# Autodesk Inventor assembly: sail(Midterm)
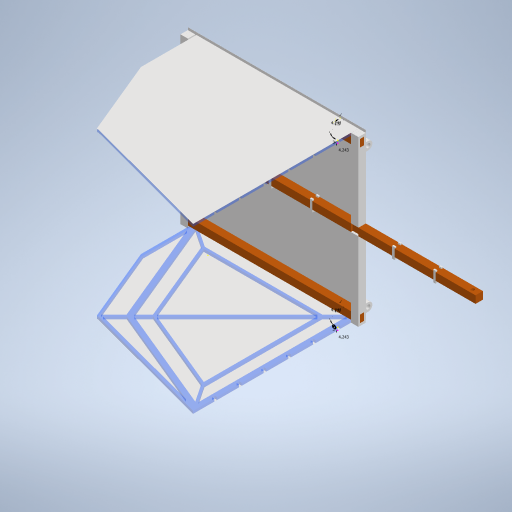
[picture p0: Inventor's stored thumbnail of the model, 512x512]
Saved by Autodesk Inventor 2024 (Build 280153000, 153)
## iProperties
Created: 2024-04-09
Part Number: sail(Midterm)
Document SubType Name: Assembly
Designer: USER
Author: USER
## Documents named in this file (11)
- E:\university\大三\大三下\機工實務\圖檔\DesignVer2\sail(Midterm).iam
- E:\university\大三\大三下\機工實務\圖檔\DesignVer2\main_Bar.ipt
- E:\university\大三\大三下\機工實務\圖檔\DesignVer2\main_Bar_3.ipt
- E:\university\大三\大三下\機工實務\圖檔\DesignVer2\Lower_Bar.ipt
- E:\university\大三\大三下\機工實務\圖檔\DesignVer2\upper_Bar.ipt
- E:\university\大三\大三下\機工實務\圖檔\DesignVer2\upper_Bar_3.ipt
- E:\university\大三\大三下\機工實務\圖檔\DesignVer2\side_Bar.ipt
- E:\university\大三\大三下\機工實務\圖檔\DesignVer2\side_sail.ipt
- E:\university\大三\大三下\機工實務\圖檔\DesignVer2\夾持器.ipt
- E:\university\大三\大三下\機工實務\圖檔\DesignVer2\帆布.ipt
- E:\university\大三\大三下\機工實務\圖檔\DesignVer2\帆布_中間.ipt
## Components (25 placed, 10 different names)
1. main_Bar:1 — 齊平:1, 齊平:2, 貼合:2, 貼合:7, 貼合:11, 貼合:26, 貼合:27, 貼合:28, 貼合:29, 貼合:33
2. main_Bar:2 — 齊平:1, 齊平:2, 齊平:3, 齊平:4, 貼合:1, 貼合:2, 貼合:5, 貼合:6, 貼合:30, 貼合:31, 貼合:32
3. main_Bar_3:1 — 齊平:3, 齊平:4, 貼合:1, 貼合:10, 齊平:13
4. Lower_Bar:1 — 齊平:5, 貼合:4, 齊平:8
5. Lower_Bar:2 — 齊平:5, 齊平:6, 貼合:3, 貼合:4, 齊平:7, 齊平:8
6. upper_Bar:1 — 貼合:9, 齊平:10, 齊平:11, 貼合:10
7. upper_Bar:2 — 貼合:8, 貼合:9, 齊平:9, 齊平:10, 齊平:11, 齊平:12, 齊平:13
8. upper_Bar_3:1 — 貼合:8, 齊平:9, 齊平:12, 貼合:11, 齊平:33
9. Lower_Bar:3 — 齊平:6, 貼合:3, 齊平:7, 貼合:5, 貼合:6, 貼合:7, 貼合:16, 貼合:17, 貼合:18, 貼合:19, 貼合:20, 貼合:21, 貼合:22, 貼合:24
10. side_Bar:1 — 貼合:12, 齊平:14, 齊平:17, 貼合:21, 齊平:22, 貼合:23, 齊平:32
11. side_Bar:2 — 貼合:12, 貼合:13, 齊平:14, 齊平:15, 齊平:16, 齊平:17, 貼合:20
12. side_Bar:3 — 貼合:13, 齊平:15, 齊平:16, 貼合:19
13. side_Bar:4 — 齊平:18, 齊平:20, 貼合:14
14. side_Bar:5 — 齊平:18, 齊平:19, 齊平:20, 齊平:21, 貼合:14, 貼合:15, 貼合:16, 貼合:18, 齊平:23
15. side_Bar:6 — 齊平:19, 齊平:21, 貼合:15, 貼合:17, 貼合:25
16. side_sail:1 — 齊平:22, 貼合:22, 貼合:23, 齊平:34, 齊平:36, 貼合:34
17. side_sail:2 — 齊平:23, 貼合:24, 貼合:25, 貼合:35, 齊平:37
18. 夾持器:1 — 齊平:24, 齊平:28, 齊平:29, 貼合:32
19. 夾持器:2 — 齊平:24, 齊平:25, 齊平:30, 貼合:31
20. 夾持器:3 — 齊平:25, 齊平:26, 齊平:31, 貼合:27, 貼合:28
21. 夾持器:4 — 齊平:26, 齊平:27, 齊平:29, 齊平:30, 齊平:31, 貼合:30
22. 夾持器:5 — 齊平:27, 貼合:26, 齊平:28, 貼合:29
23. 帆布:1 — 角度:1, 齊平:34, 齊平:35, 齊平:36, 貼合:34
24. 帆布_中間:1 — 貼合:33, 齊平:32, 齊平:33
25. 帆布:2 — 角度:1, 齊平:35, 貼合:35, 齊平:37
## Relationships (73: Flush 37, Mate 35, Angle 1)
- 齊平:1 [Flush]: main_Bar:1 ↔ main_Bar:2
- 齊平:2 [Flush]: main_Bar:1 ↔ main_Bar:2
- 齊平:3 [Flush]: main_Bar:2 ↔ main_Bar_3:1
- 齊平:4 [Flush]: main_Bar:2 ↔ main_Bar_3:1
- 貼合:1 [Mate]: main_Bar:2 ↔ main_Bar_3:1
- 貼合:2 [Mate]: main_Bar:1 ↔ main_Bar:2
- 齊平:5 [Flush]: Lower_Bar:1 ↔ Lower_Bar:2
- 齊平:6 [Flush]: Lower_Bar:2 ↔ Lower_Bar:3
- 貼合:3 [Mate]: Lower_Bar:2 ↔ Lower_Bar:3
- 貼合:4 [Mate]: Lower_Bar:1 ↔ Lower_Bar:2
- 齊平:7 [Flush]: Lower_Bar:2 ↔ Lower_Bar:3
- 齊平:8 [Flush]: Lower_Bar:1 ↔ Lower_Bar:2
- 貼合:5 [Mate]: main_Bar:2 ↔ Lower_Bar:3
- 貼合:6 [Mate]: main_Bar:2 ↔ Lower_Bar:3
- 貼合:7 [Mate]: main_Bar:1 ↔ Lower_Bar:3
- 貼合:8 [Mate]: upper_Bar:2 ↔ upper_Bar_3:1
- 貼合:9 [Mate]: upper_Bar:1 ↔ upper_Bar:2
- 齊平:9 [Flush]: upper_Bar:2 ↔ upper_Bar_3:1
- 齊平:10 [Flush]: upper_Bar:1 ↔ upper_Bar:2
- 齊平:11 [Flush]: upper_Bar:1 ↔ upper_Bar:2
- 齊平:12 [Flush]: upper_Bar:2 ↔ upper_Bar_3:1
- 貼合:10 [Mate]: main_Bar_3:1 ↔ upper_Bar:1
- 齊平:13 [Flush]: main_Bar_3:1 ↔ upper_Bar:2
- 貼合:11 [Mate]: main_Bar:1 ↔ upper_Bar_3:1
- 貼合:12 [Mate]: side_Bar:1 ↔ side_Bar:2
- 貼合:13 [Mate]: side_Bar:2 ↔ side_Bar:3
- 齊平:14 [Flush]: side_Bar:1 ↔ side_Bar:2
- 齊平:15 [Flush]: side_Bar:2 ↔ side_Bar:3
- 齊平:16 [Flush]: side_Bar:2 ↔ side_Bar:3
- 齊平:17 [Flush]: side_Bar:1 ↔ side_Bar:2
- 齊平:18 [Flush]: side_Bar:4 ↔ side_Bar:5
- 齊平:19 [Flush]: side_Bar:5 ↔ side_Bar:6
- 齊平:20 [Flush]: side_Bar:4 ↔ side_Bar:5
- 齊平:21 [Flush]: side_Bar:5 ↔ side_Bar:6
- 貼合:14 [Mate]: side_Bar:4 ↔ side_Bar:5
- 貼合:15 [Mate]: side_Bar:5 ↔ side_Bar:6
- 貼合:16 [Mate]: Lower_Bar:3 ↔ side_Bar:5
- 貼合:17 [Mate]: Lower_Bar:3 ↔ side_Bar:6
- 貼合:18 [Mate]: Lower_Bar:3 ↔ side_Bar:5
- 貼合:19 [Mate]: Lower_Bar:3 ↔ side_Bar:3
- 貼合:20 [Mate]: Lower_Bar:3 ↔ side_Bar:2
- 貼合:21 [Mate]: Lower_Bar:3 ↔ side_Bar:1
- 齊平:22 [Flush]: side_Bar:1 ↔ side_sail:1
- 貼合:22 [Mate]: Lower_Bar:3 ↔ side_sail:1
- 貼合:23 [Mate]: side_Bar:1 ↔ side_sail:1
- 齊平:23 [Flush]: side_Bar:5 ↔ side_sail:2
- 貼合:24 [Mate]: Lower_Bar:3 ↔ side_sail:2
- 貼合:25 [Mate]: side_Bar:6 ↔ side_sail:2
- 齊平:24 [Flush]: 夾持器:1 ↔ 夾持器:2
- 齊平:25 [Flush]: 夾持器:2 ↔ 夾持器:3
- 齊平:26 [Flush]: 夾持器:3 ↔ 夾持器:4
- 齊平:27 [Flush]: 夾持器:4 ↔ 夾持器:5
- 貼合:26 [Mate]: main_Bar:1 ↔ 夾持器:5
- 齊平:28 [Flush]: 夾持器:1 ↔ 夾持器:5
- 齊平:29 [Flush]: 夾持器:1 ↔ 夾持器:4
- 齊平:30 [Flush]: 夾持器:2 ↔ 夾持器:4
- 齊平:31 [Flush]: 夾持器:3 ↔ 夾持器:4
- 貼合:27 [Mate]: main_Bar:1 ↔ 夾持器:3
- 貼合:28 [Mate]: main_Bar:1 ↔ 夾持器:3
- 貼合:29 [Mate]: main_Bar:1 ↔ 夾持器:5
- 貼合:30 [Mate]: main_Bar:2 ↔ 夾持器:4
- 貼合:31 [Mate]: main_Bar:2 ↔ 夾持器:2
- 貼合:32 [Mate]: main_Bar:2 ↔ 夾持器:1
- 貼合:33 [Mate]: main_Bar:1 ↔ 帆布_中間:1
- 齊平:32 [Flush]: side_Bar:1 ↔ 帆布_中間:1
- 齊平:33 [Flush]: upper_Bar_3:1 ↔ 帆布_中間:1
- 角度:1 [Angle] (0 deg): 帆布:1 ↔ 帆布:2
- 齊平:34 [Flush]: side_sail:1 ↔ 帆布:1
- 齊平:35 [Flush]: 帆布:1 ↔ 帆布:2
- 齊平:36 [Flush]: side_sail:1 ↔ 帆布:1
- 貼合:34 [Mate]: side_sail:1 ↔ 帆布:1
- 貼合:35 [Mate]: side_sail:2 ↔ 帆布:2
- 齊平:37 [Flush]: side_sail:2 ↔ 帆布:2
